# Autodesk Inventor assembly: Zespół1
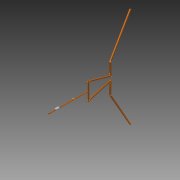
[picture p0: Inventor's stored thumbnail of the model, 180x180]
Saved by Autodesk Inventor 2015 (Build 190159000, 159)
## iProperties
Created: 2016-03-16
Part Number: Zespół1
Document SubType Name: Assembly
Designer: Arek
Author: Arek
## Documents named in this file (7)
- E:\STUDIA\SEM6\EFR\AREK PROJEKT\Zespół1.iam
- E:\STUDIA\SEM6\EFR\AREK PROJEKT\1.ipt
- E:\STUDIA\SEM6\EFR\AREK PROJEKT\2.ipt
- E:\STUDIA\SEM6\EFR\AREK PROJEKT\3.ipt
- E:\STUDIA\SEM6\EFR\AREK PROJEKT\LinearConnector.ipt
- E:\STUDIA\SEM6\EFR\AREK PROJEKT\RevolvingConnector1.ipt
- E:\STUDIA\SEM6\EFR\AREK PROJEKT\RevolvingConnector2.ipt
## Components (12 placed, 6 different names)
1. 1:1 — Walcowe:1, Sztywne:2, Sztywne:3
2. 2:1 — Obrotowe:3, Sztywne:7, Kąt:1
3. 2:2 — Obrotowe:4, Obrotowe:5, Kąt:2
4. LinearConnector:1 — Walcowe:1
5. RevolvingConnector1:1 — Sztywne:2, Obrotowe:3
6. RevolvingConnector1:2 — Sztywne:3, Obrotowe:4
7. RevolvingConnector1:3 — Sztywne:7, Obrotowe:7
8. RevolvingConnector1:4 — Obrotowe:5, Obrotowe:8
9. RevolvingConnector2:1 — Obrotowe:10
10. RevolvingConnector2:2 — Obrotowe:9
11. 3:1 — Obrotowe:7, Obrotowe:10, Kąt:1
12. 3:2 — Obrotowe:8, Obrotowe:9, Kąt:2
## Relationships (13: RevoluteJoint 7, WeldJoint 3, Angle 2, CylindricalJoint 1)
- Walcowe:1 [CylindricalJoint]: 1:1 ↔ LinearConnector:1
- Sztywne:2 [WeldJoint]: 1:1 ↔ RevolvingConnector1:1
- Sztywne:3 [WeldJoint]: 1:1 ↔ RevolvingConnector1:2
- Obrotowe:3 [RevoluteJoint]: 2:1 ↔ RevolvingConnector1:1
- Obrotowe:4 [RevoluteJoint]: 2:2 ↔ RevolvingConnector1:2
- Obrotowe:5 [RevoluteJoint]: 2:2 ↔ RevolvingConnector1:4
- Sztywne:7 [WeldJoint]: 2:1 ↔ RevolvingConnector1:3
- Obrotowe:7 [RevoluteJoint]: RevolvingConnector1:3 ↔ 3:1
- Obrotowe:8 [RevoluteJoint]: RevolvingConnector1:4 ↔ 3:2
- Obrotowe:9 [RevoluteJoint]: RevolvingConnector2:2 ↔ 3:2
- Obrotowe:10 [RevoluteJoint]: RevolvingConnector2:1 ↔ 3:1
- Kąt:1 [Angle] (-106 deg): 2:1 ↔ 3:1
- Kąt:2 [Angle] (-30 deg): 2:2 ↔ 3:2
